# Autodesk Inventor assembly: linrail_guide_asm
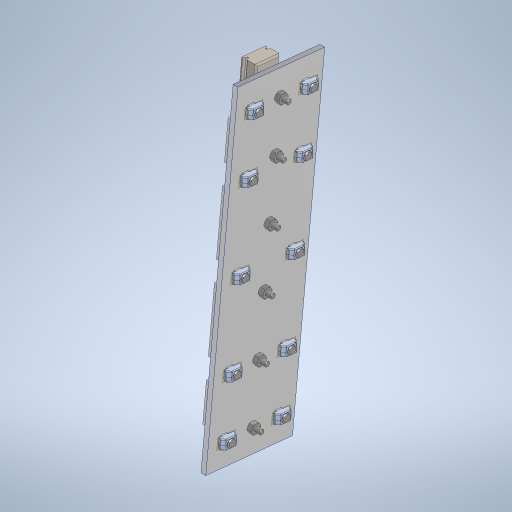
[picture p0: Inventor's stored thumbnail of the model, 512x512]
Saved by Autodesk Inventor 2024 (Build 280153000, 153)
## iProperties
Created: 2025-12-26
Part Number: linrail_guide_asm
Document SubType Name: Assembly
Designer: schar
Author: schar
## Documents named in this file (8)
- C:\Users\schar\Desktop\projectBlueprint\AMSTS\hardware\linrail_guide_asm.iam
- C:\Users\schar\Desktop\projectBlueprint\AMSTS\hardware\linrail_fix.ipt
- C:\Users\schar\Documents\Inventor\Content Center Files\R2024\en-US\ISO 4762(1)\DIN EN ISO 4762 - M5 x 8.ipt
- C:\Users\schar\Desktop\projectBlueprint\AMSTS\hardware\tnut_m5_2020.ipt
- C:\Users\schar\Desktop\projectBlueprint\AMSTS\hardware\linrail_screw_spacer.ipt
- C:\Users\schar\Desktop\projectBlueprint\AMSTS\hardware\linear_rail.ipt
- C:\Users\schar\Documents\Inventor\Content Center Files\R2024\en-US\ISO 4762(1)\DIN EN ISO 4762 - M3 x 20.ipt
- C:\Users\schar\Documents\Inventor\Content Center Files\R2024\en-US\ANSI B18.2.4.2M\ANSI B18.2.4.2M - M3x0,5 - 5,5.ipt
## Components (35 placed, 7 different names)
1. linrail_fix:1 — Rigid:1, Rigid:2, Rigid:3, Rigid:4, Rigid:5, Rigid:6, Rigid:10, Rigid:9, Rigid:8, Rigid:7, Mate:1, Mate:2, Mate:3, Mate:4, Mate:5, Mate:6, Mate:7, Mate:8, Mate:9, Mate:10, Mate:21, Mate:22, Mate:23, Mate:29, Mate:34, Mate:37, Mate:39, Mate:41, Mate:44, Mate:45, Mate:46, Mate:47, Mate:48, Mate:49
2. DIN EN ISO 4762 M5 x 8:1 — Mate:1, Mate:20
3. DIN EN ISO 4762 M5 x 8:2 — Mate:2, Mate:19
4. DIN EN ISO 4762 M5 x 8:3 — Mate:3, Mate:18
5. DIN EN ISO 4762 M5 x 8:4 — Mate:4, Mate:17
6. DIN EN ISO 4762 M5 x 8:5 — Mate:5, Mate:16
7. DIN EN ISO 4762 M5 x 8:6 — Mate:6, Mate:15
8. DIN EN ISO 4762 M5 x 8:7 — Mate:7, Mate:14
9. DIN EN ISO 4762 M5 x 8:8 — Mate:8, Mate:13
10. DIN EN ISO 4762 M5 x 8:9 — Mate:9, Mate:12
11. DIN EN ISO 4762 M5 x 8:10 — Mate:10, Mate:11
12. tnut_m5_2020:1 — Rigid:1, Mate:11
13. tnut_m5_2020:2 — Rigid:2, Mate:12
14. tnut_m5_2020:3 — Rigid:3, Mate:13
15. tnut_m5_2020:4 — Rigid:4, Mate:14
16. tnut_m5_2020:5 — Rigid:5, Mate:15
17. tnut_m5_2020:6 — Rigid:7, Mate:16
18. tnut_m5_2020:7 — Rigid:8, Mate:17
19. tnut_m5_2020:8 — Rigid:9, Mate:18
20. tnut_m5_2020:9 — Rigid:10, Mate:19
21. tnut_m5_2020:10 — Rigid:6, Mate:20
22. linrail_screw_spacer:1 — Mate:21, Mate:22, Mate:23, Mate:30, Mate:35
23. DIN EN ISO 4762 M3 x 20:1 — Mate:33, Mate:34, Mate:55
24. DIN EN ISO 4762 M3 x 20:2 — Mate:29, Mate:31, Mate:32, Mate:54
25. DIN EN ISO 4762 M3 x 20:3 — Mate:36, Mate:37, Mate:53
26. DIN EN ISO 4762 M3 x 20:4 — Mate:38, Mate:39, Mate:52
27. DIN EN ISO 4762 M3 x 20:5 — Mate:40, Mate:41, Mate:51
28. DIN EN ISO 4762 M3 x 20:6 — Mate:42, Mate:43, Mate:50
29. linear_rail:1 — Mate:30, Mate:31, Mate:32, Mate:33, Mate:35, Mate:36, Mate:38, Mate:40, Mate:42, Mate:43
30. ANSI B18.2.4.2M M3x0,5:1 — Mate:44, Mate:55
31. ANSI B18.2.4.2M M3x0,5:2 — Mate:45, Mate:54
32. ANSI B18.2.4.2M M3x0,5:3 — Mate:46, Mate:53
33. ANSI B18.2.4.2M M3x0,5:4 — Mate:47, Mate:52
34. ANSI B18.2.4.2M M3x0,5:5 — Mate:48, Mate:51
35. ANSI B18.2.4.2M M3x0,5:6 — Mate:49, Mate:50
## Relationships (60: Mate 50, WeldJoint 10)
- Rigid:1 [WeldJoint] (0.159 mm): linrail_fix:1 ↔ tnut_m5_2020:1
- Rigid:2 [WeldJoint] (0.159 mm): linrail_fix:1 ↔ tnut_m5_2020:2
- Rigid:3 [WeldJoint] (0.159 mm): linrail_fix:1 ↔ tnut_m5_2020:3
- Rigid:4 [WeldJoint] (0.159 mm): linrail_fix:1 ↔ tnut_m5_2020:4
- Rigid:5 [WeldJoint] (0.159 mm): linrail_fix:1 ↔ tnut_m5_2020:5
- Rigid:6 [WeldJoint] (0.159 mm): linrail_fix:1 ↔ tnut_m5_2020:10
- Rigid:10 [WeldJoint] (0.159 mm): linrail_fix:1 ↔ tnut_m5_2020:9
- Rigid:9 [WeldJoint] (0.159 mm): linrail_fix:1 ↔ tnut_m5_2020:8
- Rigid:8 [WeldJoint] (0.159 mm): linrail_fix:1 ↔ tnut_m5_2020:7
- Rigid:7 [WeldJoint] (0.159 mm): linrail_fix:1 ↔ tnut_m5_2020:6
- Mate:1: linrail_fix:1 ↔ DIN EN ISO 4762 M5 x 8:1
- Mate:2: linrail_fix:1 ↔ DIN EN ISO 4762 M5 x 8:2
- Mate:3: linrail_fix:1 ↔ DIN EN ISO 4762 M5 x 8:3
- Mate:4: linrail_fix:1 ↔ DIN EN ISO 4762 M5 x 8:4
- Mate:5: linrail_fix:1 ↔ DIN EN ISO 4762 M5 x 8:5
- Mate:6: linrail_fix:1 ↔ DIN EN ISO 4762 M5 x 8:6
- Mate:7: linrail_fix:1 ↔ DIN EN ISO 4762 M5 x 8:7
- Mate:8: linrail_fix:1 ↔ DIN EN ISO 4762 M5 x 8:8
- Mate:9: linrail_fix:1 ↔ DIN EN ISO 4762 M5 x 8:9
- Mate:10: linrail_fix:1 ↔ DIN EN ISO 4762 M5 x 8:10
- Mate:11: DIN EN ISO 4762 M5 x 8:10 ↔ tnut_m5_2020:1
- Mate:12: DIN EN ISO 4762 M5 x 8:9 ↔ tnut_m5_2020:2
- Mate:13: DIN EN ISO 4762 M5 x 8:8 ↔ tnut_m5_2020:3
- Mate:14: DIN EN ISO 4762 M5 x 8:7 ↔ tnut_m5_2020:4
- Mate:15: DIN EN ISO 4762 M5 x 8:6 ↔ tnut_m5_2020:5
- Mate:16: DIN EN ISO 4762 M5 x 8:5 ↔ tnut_m5_2020:6
- Mate:17: DIN EN ISO 4762 M5 x 8:4 ↔ tnut_m5_2020:7
- Mate:18: DIN EN ISO 4762 M5 x 8:3 ↔ tnut_m5_2020:8
- Mate:19: DIN EN ISO 4762 M5 x 8:2 ↔ tnut_m5_2020:9
- Mate:20: DIN EN ISO 4762 M5 x 8:1 ↔ tnut_m5_2020:10
- Mate:21: linrail_fix:1 ↔ linrail_screw_spacer:1
- Mate:22: linrail_fix:1 ↔ linrail_screw_spacer:1
- Mate:23: linrail_fix:1 ↔ linrail_screw_spacer:1
- Mate:29: linrail_fix:1 ↔ DIN EN ISO 4762 M3 x 20:2
- Mate:30: linrail_screw_spacer:1 ↔ linear_rail:1
- Mate:31: DIN EN ISO 4762 M3 x 20:2 ↔ linear_rail:1
- Mate:32: DIN EN ISO 4762 M3 x 20:2 ↔ linear_rail:1
- Mate:33: DIN EN ISO 4762 M3 x 20:1 ↔ linear_rail:1
- Mate:34: linrail_fix:1 ↔ DIN EN ISO 4762 M3 x 20:1
- Mate:35: linrail_screw_spacer:1 ↔ linear_rail:1
- Mate:36: DIN EN ISO 4762 M3 x 20:3 ↔ linear_rail:1
- Mate:37: linrail_fix:1 ↔ DIN EN ISO 4762 M3 x 20:3
- Mate:38: DIN EN ISO 4762 M3 x 20:4 ↔ linear_rail:1
- Mate:39: linrail_fix:1 ↔ DIN EN ISO 4762 M3 x 20:4
- Mate:40: DIN EN ISO 4762 M3 x 20:5 ↔ linear_rail:1
- Mate:41: linrail_fix:1 ↔ DIN EN ISO 4762 M3 x 20:5
- Mate:42: DIN EN ISO 4762 M3 x 20:6 ↔ linear_rail:1
- Mate:43: DIN EN ISO 4762 M3 x 20:6 ↔ linear_rail:1
- Mate:44: linrail_fix:1 ↔ ANSI B18.2.4.2M M3x0,5:1
- Mate:45: linrail_fix:1 ↔ ANSI B18.2.4.2M M3x0,5:2
- Mate:46: linrail_fix:1 ↔ ANSI B18.2.4.2M M3x0,5:3
- Mate:47: linrail_fix:1 ↔ ANSI B18.2.4.2M M3x0,5:4
- Mate:48: linrail_fix:1 ↔ ANSI B18.2.4.2M M3x0,5:5
- Mate:49: linrail_fix:1 ↔ ANSI B18.2.4.2M M3x0,5:6
- Mate:50: DIN EN ISO 4762 M3 x 20:6 ↔ ANSI B18.2.4.2M M3x0,5:6
- Mate:51: DIN EN ISO 4762 M3 x 20:5 ↔ ANSI B18.2.4.2M M3x0,5:5
- Mate:52: DIN EN ISO 4762 M3 x 20:4 ↔ ANSI B18.2.4.2M M3x0,5:4
- Mate:53: DIN EN ISO 4762 M3 x 20:3 ↔ ANSI B18.2.4.2M M3x0,5:3
- Mate:54: DIN EN ISO 4762 M3 x 20:2 ↔ ANSI B18.2.4.2M M3x0,5:2
- Mate:55: DIN EN ISO 4762 M3 x 20:1 ↔ ANSI B18.2.4.2M M3x0,5:1
